# Autodesk Inventor assembly: Motor_Node
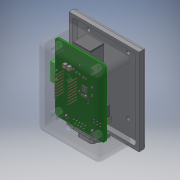
[picture p0: Inventor's stored thumbnail of the model, 180x180]
Saved by Autodesk Inventor 2019.4 (Build 234330000, 330)
## iProperties
Created: 2019-12-12
Part Number: Motor_Node
Document SubType Name: Assembly
Designer: Jorian Brusind
Author: Jorian Brusind
## Documents named in this file (4)
- C:\Users\Jorian Bruslind\Documents\GitHub\ECE44x_Senior_Design\Design files\Delta Robot Arm\Inventor Files\Custom_Delta\Motor_Node.iam
- C:\Users\Jorian Bruslind\Documents\GitHub\ECE44x_Senior_Design\Design files\Delta Robot Arm\Inventor Files\Custom_Delta\Motor_Node_box.ipt
- C:\Users\Jorian Bruslind\Documents\GitHub\ECE44x_Senior_Design\Design files\Delta Robot Arm\Inventor Files\Custom_Delta\Motor_Node_top.ipt
- C:\Users\Jorian Bruslind\Documents\GitHub\ECE44x_Senior_Design\Design files\Delta Robot Arm\PCB Files\Stepper Motor Driver PCB\ExportSTEP\TMC2209_PCB.iam
## Components (3 placed, 3 different names)
1. Motor_Node_box:1 — Mate:19, Mate:20, Mate:21, Mate:22, Mate:23
2. Motor_Node_top:1 — Mate:22, Mate:23
3. TMC2209_PCB:1 [sub-assembly] — Mate:19, Mate:20, Mate:21
## Relationships (5: Mate 5)
- Mate:19: Motor_Node_box:1 ↔ TMC2209_PCB:1
- Mate:20: Motor_Node_box:1 ↔ TMC2209_PCB:1
- Mate:21: Motor_Node_box:1 ↔ TMC2209_PCB:1
- Mate:22: Motor_Node_box:1 ↔ Motor_Node_top:1
- Mate:23: Motor_Node_box:1 ↔ Motor_Node_top:1
